# Autodesk Inventor assembly: steadier_grabber
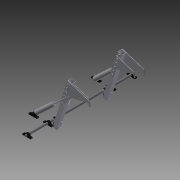
[picture p0: Inventor's stored thumbnail of the model, 180x180]
Saved by Autodesk Inventor 2011 (Build 150239000, 239)
## iProperties
Created: 2013-01-19
Part Number: steadier_grabber
Document SubType Name: Assembly
Designer: Christopher
Author: Christopher
## Documents named in this file (6)
- F:\Users\Christopher\Documents\GitHub\2013CAD\2013 robot\forklift\Pneumatics and frame grabbers\steadier_grabber.iam
- F:\Users\Christopher\Documents\GitHub\2013CAD\2013 robot\forklift\Pneumatics and frame grabbers\right_grabber.iam
- F:\Users\Christopher\Documents\GitHub\2013CAD\2013 robot\forklift\Pneumatics and frame grabbers\left_grabber.iam
- F:\Users\Christopher\Documents\GitHub\2013CAD\2013 robot\forklift\frame parts\0.5unkeyedaxle_26.ipt
- F:\Users\Christopher\Documents\GitHub\2013CAD\2013 robot\forklift\Misc parts\.5inch_side_bearing.ipt
- F:\Users\Christopher\Documents\GitHub\2013CAD\2013 robot\forklift\Pneumatics and frame grabbers\temp_cylinder_.1inch_4stroke.ipt
## Components (11 placed, 5 different names)
1. right_grabber:1 [sub-assembly] — Insert:5, Flush:4, Insert:10
2. left_grabber:1 [sub-assembly] — Insert:6, Flush:4
3. 0.5unkeyedaxle_26:1 — Insert:1, Insert:2, Insert:3, Insert:4, Insert:5, Insert:6
4. .5inch_side_bearing:1 — Insert:1, Flush:2
5. .5inch_side_bearing:2 — Insert:2, Flush:1, Flush:2, Mate:1, Flush:5, Flush:6
6. .5inch_side_bearing:3 — Insert:3, Flush:3
7. .5inch_side_bearing:4 — Insert:4, Flush:1, Flush:3, Flush:7, Flush:8, Mate:2
8. .5inch_side_bearing:5 — Mate:1, Flush:5, Flush:6, Insert:9
9. .5inch_side_bearing:6 — Flush:7, Flush:8, Mate:2, Insert:8
10. temp_cylinder_.1inch_4stroke:1 — Insert:9, Flush:9, Insert:10
11. temp_cylinder_.1inch_4stroke:2 — Insert:8, Flush:9
## Relationships (20: Insert 9, Flush 9, Mate 2)
- Insert:1 (6.35 mm): 0.5unkeyedaxle_26:1 ↔ .5inch_side_bearing:1
- Insert:2 (133.35 mm): 0.5unkeyedaxle_26:1 ↔ .5inch_side_bearing:2
- Insert:3 (6.35 mm): 0.5unkeyedaxle_26:1 ↔ .5inch_side_bearing:3
- Insert:4 (133.35 mm): 0.5unkeyedaxle_26:1 ↔ .5inch_side_bearing:4
- Flush:1: .5inch_side_bearing:2 ↔ .5inch_side_bearing:4
- Flush:2: .5inch_side_bearing:1 ↔ .5inch_side_bearing:2
- Flush:3: .5inch_side_bearing:3 ↔ .5inch_side_bearing:4
- Insert:5 (165.1 mm): right_grabber:1 ↔ 0.5unkeyedaxle_26:1
- Insert:6 (165.1 mm): left_grabber:1 ↔ 0.5unkeyedaxle_26:1
- Flush:4: right_grabber:1 ↔ left_grabber:1
- Mate:1 (38.1 mm): .5inch_side_bearing:2 ↔ .5inch_side_bearing:5
- Flush:5: .5inch_side_bearing:2 ↔ .5inch_side_bearing:5
- Flush:6: .5inch_side_bearing:2 ↔ .5inch_side_bearing:5
- Flush:7: .5inch_side_bearing:4 ↔ .5inch_side_bearing:6
- Flush:8: .5inch_side_bearing:4 ↔ .5inch_side_bearing:6
- Mate:2 (38.1 mm): .5inch_side_bearing:4 ↔ .5inch_side_bearing:6
- Insert:8: .5inch_side_bearing:6 ↔ temp_cylinder_.1inch_4stroke:2
- Insert:9: .5inch_side_bearing:5 ↔ temp_cylinder_.1inch_4stroke:1
- Flush:9: temp_cylinder_.1inch_4stroke:1 ↔ temp_cylinder_.1inch_4stroke:2
- Insert:10 (-6.35 mm): right_grabber:1 ↔ temp_cylinder_.1inch_4stroke:1
